# Autodesk Inventor assembly: khurramf_Version2_Assembly
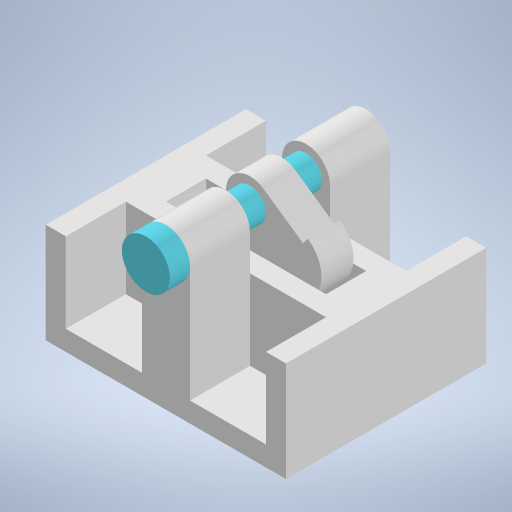
[picture p0: Inventor's stored thumbnail of the model, 512x512]
Saved by Autodesk Inventor 2024 (Build 280153000, 153)
## iProperties
Created: 2024-01-30
Part Number: khurramf_Version2_Assembly
Document SubType Name: Assembly
Designer: furqa
Author: furqa
## Documents named in this file (4)
- C:\Users\furqa\Desktop\CAD Files\Winter 1P13\GraphicsFinal_khurramf_Version2\khurramf_Version2_Assembly.iam
- C:\Users\furqa\Desktop\CAD Files\Winter 1P13\GraphicsFinal_khurramf_Version2\khurramf_Version2_Base.ipt
- C:\Users\furqa\Desktop\CAD Files\Winter 1P13\GraphicsFinal_khurramf_Version2\khurramf_Version2_Axle.ipt
- C:\Users\furqa\Desktop\CAD Files\Winter 1P13\GraphicsFinal_khurramf_Version2\khurramf_Version2_Swing.ipt
## Components (3 placed, 3 different names)
1. khurramf_Version2_Base:1 — Mate:1, Mate:2, Flush:1, Mate:3, Angle:1
2. khurramf_Version2_Axle:1 — Mate:2, Flush:1
3. khurramf_Version2_Swing:1 — Mate:1, Mate:3, Angle:1
## Relationships (5: Mate 3, Flush 1, Angle 1)
- Mate:1: khurramf_Version2_Base:1 ↔ khurramf_Version2_Swing:1
- Mate:2: khurramf_Version2_Base:1 ↔ khurramf_Version2_Axle:1
- Flush:1: khurramf_Version2_Base:1 ↔ khurramf_Version2_Axle:1
- Mate:3 (1 mm): khurramf_Version2_Base:1 ↔ khurramf_Version2_Swing:1
- Angle:1 (0 deg): khurramf_Version2_Base:1 ↔ khurramf_Version2_Swing:1
## Named parameters: Finish1_Area = 15.5823, Finish2_Area = 1.13097
note: some values were not read from the file. Shown as the stored number, unit unknown: "Finish1_Area", "Finish2_Area".
